# Autodesk Inventor assembly: FInal Setup_3
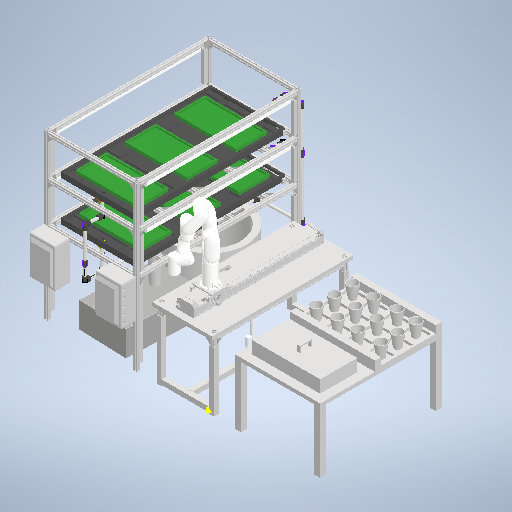
[picture p0: Inventor's stored thumbnail of the model, 512x512]
Saved by Autodesk Inventor 2025 (Build 290162000, 162)
## iProperties
Created: 2024-07-11
Part Number: FInal Setup_3
Document SubType Name: Assembly
Designer: User
Author: User
## Documents named in this file (4)
- C:\Users\User\OneDrive\Documents\FYP\Inventor_Designs\Submission_1\Setups\FInal Setup_3.iam
- C:\Users\User\OneDrive\Documents\FYP\Inventor_Designs\Setups\Setup_1_part_4.iam
- C:\Users\User\OneDrive\Documents\FYP\Inventor_Designs\Submission_1\Assembly Rack_Submission.iam
- C:\Users\User\OneDrive\Documents\FYP\Inventor_Designs\Setups\Table_Setup_2.iam
## Components (3 placed, 3 different names)
1. Setup_1_part_4:1 [sub-assembly] — Mate:2, Flush:1, Flush:2
2. Assembly Rack_Submission:1 [sub-assembly] — Flush:1, Flush:2
3. Table_Setup_2:1 [sub-assembly] — Mate:2
## Relationships (3: Flush 2, Mate 1)
- Mate:2: Setup_1_part_4:1 ↔ Table_Setup_2:1
- Flush:1: Setup_1_part_4:1 ↔ Assembly Rack_Submission:1
- Flush:2: Setup_1_part_4:1 ↔ Assembly Rack_Submission:1
